# Autodesk Inventor assembly: BoltWasher4x18
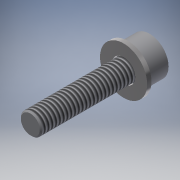
[picture p0: Inventor's stored thumbnail of the model, 180x180]
Saved by Autodesk Inventor 2016 (Build 200138000, 138)
## iProperties
Category: Hardware
Created: 2015-03-19
Part Number: BoltWasher4x18
Document SubType Name: Assembly
Designer: Jack
Mass: 0.640671 g
Surface Area: 5.44984 cm^2
Volume: 0.389092 cm^3
Density: 1.64658 g/cm^3
Vendor: McMaster Carr
Author: Jack
Title: Bolt + Washer 4x18
## Documents named in this file (3)
- C:\Users\Jack\ownCloud\Projects\CrossBot\InventorModel\Hardware\BoltWashers\BoltWasher4\BoltWasher4x18.iam
- C:\Users\Jack\ownCloud\Projects\CrossBot\InventorModel\Hardware\Bolts\SHCS\SHCS4\SHCS4x18.ipt
- C:\Users\Jack\ownCloud\Projects\CrossBot\InventorModel\Hardware\Wahsers\M4Washer.ipt
## Components (2 placed, 2 different names)
1. SHCS4x18:1 — Mate:1, Mate:2
2. M4Washer:1 — Mate:1, Mate:2
## Relationships (2: Mate 2)
- Mate:1: SHCS4x18:1 ↔ M4Washer:1
- Mate:2: SHCS4x18:1 ↔ M4Washer:1
